# Autodesk Inventor assembly: friedEggsUnit
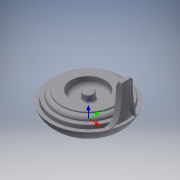
[picture p0: Inventor's stored thumbnail of the model, 180x180]
Saved by Autodesk Inventor 2016 (Build 200138000, 138)
## iProperties
Created: 2014-07-25
Part Number: friedEggsUnit
Document SubType Name: Assembly
Designer: hatakeyama
Author: hatakeyama
## Documents named in this file (3)
- \\sun\nei\nei\others\cad\enviromentModel\prepareBreakfast\friedEggsUnit.iam
- \\sun\nei\nei\others\cad\enviromentModel\prepareBreakfast\friedEggsUnit.ipt
- \\sun\nei\nei\others\cad\enviromentModel\prepareBreakfast\friedEggsCover.ipt
## Components (2 placed, 2 different names)
1. friedEggsUnit:1 — メイト:1, メイト:2, 挿入:1
2. friedEggsCover:1 — 挿入:1
## Relationships (3: Mate 2, Insert 1)
- メイト:1 [Mate]: friedEggsUnit:1
- メイト:2 [Mate]: friedEggsUnit:1
- 挿入:1 [Insert]: friedEggsUnit:1 ↔ friedEggsCover:1
